# Autodesk Inventor assembly: !drivebay
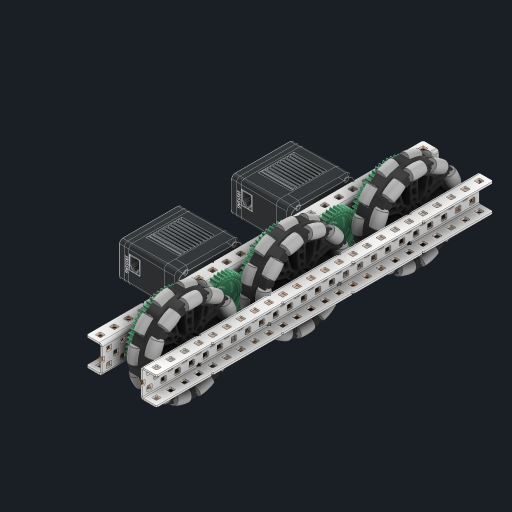
[picture p0: Inventor's stored thumbnail of the model, 512x512]
Saved by Autodesk Inventor 2024 (Build 280153000, 153)
## iProperties
Created: 2024-06-23
Part Number: !drivebay
Document SubType Name: Assembly
Designer: Averey Ku
Author: Averey Ku
## Documents named in this file (9)
- D:\vex_robotics_high_stakes\hardware\cad\prog_chassis\drivebay\!drivebay.iam
- D:\vex_robotics_high_stakes\hardware\cad\VEX-CAD-Inventor\Structure\C Channel\Aluminum 1x2x1\Alu C 1x2x1x24.ipt
- D:\vex_robotics_high_stakes\hardware\cad\VEX-CAD-Inventor\Motion\Wheels\Omni Wheel\3.25 Omni AS, No Insert.iam
- D:\vex_robotics_high_stakes\hardware\cad\VEX-CAD-Inventor\Motion\Wheels\Omni Wheel.iam
- D:\vex_robotics_high_stakes\hardware\cad\VEX-CAD-Inventor\Motion\Gears\LS 60T Gear.ipt
- D:\vex_robotics_high_stakes\hardware\cad\VEX-CAD-Inventor\Motion\Gears\LS 36T Gear.ipt
- D:\vex_robotics_high_stakes\hardware\cad\VEX-CAD-Inventor\Structure\C Channel\Aluminum 1x2x1\Alu C 1x2x1x5.ipt
- D:\vex_robotics_high_stakes\hardware\cad\VEX-CAD-Inventor\Electronics\Motors with Screws\SteelM-StarS.iam
- D:\vex_robotics_high_stakes\hardware\cad\VEX-CAD-Inventor\Electronics\Motors with Screws.iam
## Components (13 placed, 6 different names)
1. Alu C 1x2x1x24:1 — Insert:1, Insert:2, Insert:3, Mate:1, Mate:2, Insert:7, Mate:3
2. 3.25 Omni AS, No Insert:1 [sub-assembly] — Insert:1, Insert:4
3. 3.25 Omni AS, No Insert:2 [sub-assembly] — Insert:2, Insert:5
4. 3.25 Omni AS, No Insert:3 [sub-assembly] — Insert:3, Insert:6
5. LS 60T Gear:1 — Insert:4
6. LS 60T Gear:2 — Insert:5, Flush:1
7. LS 60T Gear:3 — Insert:6, Flush:2
8. LS 36T Gear:1 — Mate:1, Flush:1
9. LS 36T Gear:2 — Mate:2, Flush:2
10. Alu C 1x2x1x24:2 — Insert:8, Mate:4, Insert:9, Mate:5, Insert:10, Mate:6
11. Alu C 1x2x1x5:1 — Insert:7, Mate:3, Insert:8, Mate:4
12. SteelM-StarS:1 [sub-assembly] — Insert:9, Mate:5
13. SteelM-StarS:3 [sub-assembly] — Insert:10, Mate:6
## Relationships (18: Insert 10, Mate 6, Flush 2)
- Insert:1 (6.35 mm): Alu C 1x2x1x24:1 ↔ 3.25 Omni AS, No Insert:1
- Insert:2 (6.35 mm): Alu C 1x2x1x24:1 ↔ 3.25 Omni AS, No Insert:2
- Insert:3 (6.35 mm): Alu C 1x2x1x24:1 ↔ 3.25 Omni AS, No Insert:3
- Insert:4 (4.7625 mm): 3.25 Omni AS, No Insert:1 ↔ LS 60T Gear:1
- Insert:5 (4.7625 mm): 3.25 Omni AS, No Insert:2 ↔ LS 60T Gear:2
- Insert:6 (4.7625 mm): 3.25 Omni AS, No Insert:3 ↔ LS 60T Gear:3
- Mate:1: Alu C 1x2x1x24:1 ↔ LS 36T Gear:1
- Flush:1: LS 60T Gear:2 ↔ LS 36T Gear:1
- Mate:2: Alu C 1x2x1x24:1 ↔ LS 36T Gear:2
- Flush:2: LS 60T Gear:3 ↔ LS 36T Gear:2
- Insert:7: Alu C 1x2x1x24:1 ↔ Alu C 1x2x1x5:1
- Mate:3: Alu C 1x2x1x24:1 ↔ Alu C 1x2x1x5:1
- Insert:8: Alu C 1x2x1x24:2 ↔ Alu C 1x2x1x5:1
- Mate:4: Alu C 1x2x1x24:2 ↔ Alu C 1x2x1x5:1
- Insert:9: Alu C 1x2x1x24:2 ↔ SteelM-StarS:1
- Mate:5: Alu C 1x2x1x24:2 ↔ SteelM-StarS:1
- Insert:10: Alu C 1x2x1x24:2 ↔ SteelM-StarS:3
- Mate:6: Alu C 1x2x1x24:2 ↔ SteelM-StarS:3
